# Autodesk Inventor assembly: base+motors
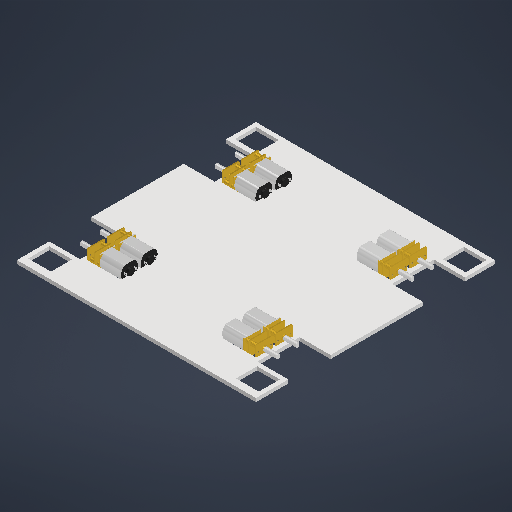
[picture p0: Inventor's stored thumbnail of the model, 512x512]
Saved by Autodesk Inventor 2026.2 (Build 302298010, 298A)
## iProperties
Created: 2026-03-30
Part Number: base+motors
Document SubType Name: Assembly
Designer: karol
Author: karol
## Documents named in this file (3)
- C:\Users\karol\OneDrive\Desktop\robo\bolt\cad\assembly\base+motors.iam
- C:\Users\karol\OneDrive\Desktop\robo\bolt\cad\ready parts\base.ipt
- C:\Users\karol\OneDrive\Desktop\robo\bolt\cad\ready parts\Pololu #2218 Micro Metal Gearmotor HP.ipt
## Components (9 placed, 2 different names)
1. base:2 — Mate:1, Mate:2, Mate:3, Mate:4, Mate:5, Mate:6, Mate:7, Mate:8, Mate:9, Mate:10, Mate:11, Mate:12, Mate:13, Mate:14, Mate:15, Mate:16
2. Pololu #2218 Micro Metal Gearmotor HP:1 — Mate:3, Mate:4
3. Pololu #2218 Micro Metal Gearmotor HP:2 — Mate:5, Mate:6
4. Pololu #2218 Micro Metal Gearmotor HP:3 — Mate:7, Mate:8
5. Pololu #2218 Micro Metal Gearmotor HP:4 — Mate:1, Mate:2
6. Pololu #2218 Micro Metal Gearmotor HP:5 — Mate:13, Mate:14
7. Pololu #2218 Micro Metal Gearmotor HP:6 — Mate:15, Mate:16
8. Pololu #2218 Micro Metal Gearmotor HP:7 — Mate:11, Mate:12
9. Pololu #2218 Micro Metal Gearmotor HP:8 — Mate:9, Mate:10
## Relationships (16: Mate 16)
- Mate:1: base:2 ↔ Pololu #2218 Micro Metal Gearmotor HP:4
- Mate:2: base:2 ↔ Pololu #2218 Micro Metal Gearmotor HP:4
- Mate:3: base:2 ↔ Pololu #2218 Micro Metal Gearmotor HP:1
- Mate:4: base:2 ↔ Pololu #2218 Micro Metal Gearmotor HP:1
- Mate:5: base:2 ↔ Pololu #2218 Micro Metal Gearmotor HP:2
- Mate:6: base:2 ↔ Pololu #2218 Micro Metal Gearmotor HP:2
- Mate:7: base:2 ↔ Pololu #2218 Micro Metal Gearmotor HP:3
- Mate:8: base:2 ↔ Pololu #2218 Micro Metal Gearmotor HP:3
- Mate:9: base:2 ↔ Pololu #2218 Micro Metal Gearmotor HP:8
- Mate:10: base:2 ↔ Pololu #2218 Micro Metal Gearmotor HP:8
- Mate:11: base:2 ↔ Pololu #2218 Micro Metal Gearmotor HP:7
- Mate:12: base:2 ↔ Pololu #2218 Micro Metal Gearmotor HP:7
- Mate:13: base:2 ↔ Pololu #2218 Micro Metal Gearmotor HP:5
- Mate:14: base:2 ↔ Pololu #2218 Micro Metal Gearmotor HP:5
- Mate:15: base:2 ↔ Pololu #2218 Micro Metal Gearmotor HP:6
- Mate:16: base:2 ↔ Pololu #2218 Micro Metal Gearmotor HP:6
